# Autodesk Inventor assembly: arm_assembly
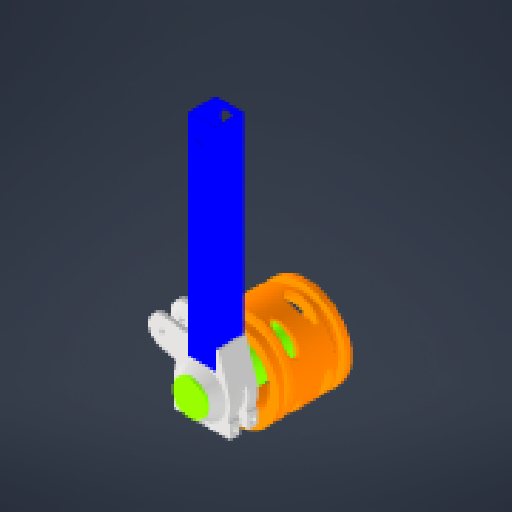
[picture p0: Inventor's stored thumbnail of the model, 512x512]
Saved by Autodesk Inventor 2024 (Build 280153000, 153)
## iProperties
Created: 2023-09-26
Part Number: arm_assembly
Document SubType Name: Assembly
Designer: user
Author: user
## Documents named in this file (5)
- D:\Docs\Robot\3d_v2\machine_body\arm_assembly_l.iam
- D:\Docs\Robot\3d_v2\base\arm.ipt
- D:\Docs\Robot\3d_v2\machine_body\arm_assembly\motor_holder.ipt
- D:\Docs\Robot\3d_v2\machine_body\wheel_assembly\wheel.ipt
- D:\Docs\Robot\3d_v2\default_components\motor.ipt
## Components (4 placed, 4 different names)
1. arm:1 — Совмещение:1, Совмещение:2, Совмещение:3, Совмещение:4, Совмещение:5, Совмещение:6, Совмещение:10
2. wheel:2 — Вставка:1, Совмещение:10
3. motor:1 — Совмещение:9, Вставка:1
4. motor_holder:1 — Совмещение:4, Совмещение:5, Совмещение:6, Совмещение:9
## Relationships (9: Mate 8, Insert 1)
- Совмещение:1 [Mate]: arm:1
- Совмещение:2 [Mate]: arm:1
- Совмещение:3 [Mate]: arm:1
- Совмещение:4 [Mate]: arm:1 ↔ motor_holder:1
- Совмещение:5 [Mate]: arm:1 ↔ motor_holder:1
- Совмещение:6 [Mate]: arm:1 ↔ motor_holder:1
- Совмещение:9 [Mate]: motor:1 ↔ motor_holder:1
- Вставка:1 [Insert]: wheel:2 ↔ motor:1
- Совмещение:10 [Mate] (3 mm): arm:1 ↔ wheel:2
